# Autodesk Inventor assembly: Assembly1
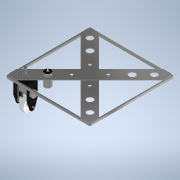
[picture p0: Inventor's stored thumbnail of the model, 180x180]
Saved by Autodesk Inventor 2020 (Build 240168000, 168)
## iProperties
Created: 2022-07-06
Part Number: Assembly1
Document SubType Name: Assembly
Designer: karimi2
Author: karimi2
## Documents named in this file (4)
- C:\Users\karimi2\Documents\PROJECT\src\Assembly1.iam
- C:\Users\karimi2\Documents\PROJECT\src\Chassis.ipt
- C:\Users\karimi2\Documents\PROJECT\src\Wheel Assembly.iam
- C:\Users\karimi2\Documents\PROJECT\src\GearedDCmotor.ipt
## Components (3 placed, 3 different names)
1. Chassis:1 — Mate:1, Rotational:1, Mate:2, Rigid:1
2. Wheel Assembly:1 [sub-assembly] — Mate:1, Rotational:1
3. GearedDCmotor:1 — Mate:2, Rigid:1
## Relationships (4: Mate 2, RevoluteJoint 1, WeldJoint 1)
- Mate:1: Chassis:1 ↔ Wheel Assembly:1
- Rotational:1 [RevoluteJoint] (-3.5 mm): Chassis:1 ↔ Wheel Assembly:1
- Mate:2: Chassis:1 ↔ GearedDCmotor:1
- Rigid:1 [WeldJoint] (-6 mm): Chassis:1 ↔ GearedDCmotor:1
